# Autodesk Inventor assembly: Pod_pull
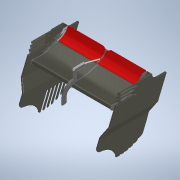
[picture p0: Inventor's stored thumbnail of the model, 180x180]
Saved by Autodesk Inventor 2022 (Build 260153000, 153)
## iProperties
Created: 2022-07-04
Part Number: Pod_pull
Document SubType Name: Assembly
Designer: corra
Author: corra
## Documents named in this file (7)
- C:\Users\corra\Desktop\Università Trento\Master degree\1st year\Mechatronic system simulation\Module 2\DRS_Project\File Cad 3D\final\assembly.iam
- C:\Users\corra\Desktop\Università Trento\Master degree\1st year\Mechatronic system simulation\Module 2\DRS_Project\File Cad 3D\final\flap.ipt
- C:\Users\corra\Desktop\Università Trento\Master degree\1st year\Mechatronic system simulation\Module 2\DRS_Project\File Cad 3D\final\main_plate.ipt
- C:\Users\corra\Desktop\Università Trento\Master degree\1st year\Mechatronic system simulation\Module 2\DRS_Project\File Cad 3D\final\pod.ipt
- C:\Users\corra\Desktop\Università Trento\Master degree\1st year\Mechatronic system simulation\Module 2\DRS_Project\File Cad 3D\final\actuator.ipt
- C:\Users\corra\Documents\Inventor\Content Center Files\R2022\it-IT\BS 1804\BS 1804-2 - 5 x 12.ipt
- C:\Users\corra\Documents\Inventor\Content Center Files\R2022\it-IT\BS 1804\BS 1804-2 - 3 x 10.ipt
## Components (6 placed, 6 different names)
1. flap:1 — Coincidente:1, Coincidente:2, Coincidente:4, Allineato:4, Coincidente:14, Coincidente:15, Allineato:5
2. main_plate:1 — Coincidente:1, Coincidente:2, Coincidente:5, Allineato:3, Coincidente:13
3. pod:1 — Coincidente:4, Coincidente:11, Coincidente:14
4. actuator:1 — Coincidente:5, Coincidente:10, Coincidente:12, Coincidente:13
5. BS 1804 : Parte 2 3 x 10:1 — Coincidente:10, Coincidente:11, Coincidente:12
6. BS 1804 : Parte 2 5 x 12:2 — Coincidente:15, Allineato:5
## Relationships (13: Mate 10, Flush 3)
- Coincidente:1 [Mate]: flap:1 ↔ main_plate:1
- Coincidente:2 [Mate]: flap:1 ↔ main_plate:1
- Coincidente:4 [Mate]: flap:1 ↔ pod:1
- Coincidente:5 [Mate]: main_plate:1 ↔ actuator:1
- Allineato:3 [Flush]: main_plate:1
- Allineato:4 [Flush]: flap:1
- Coincidente:10 [Mate]: actuator:1 ↔ BS 1804 : Parte 2 3 x 10:1
- Coincidente:11 [Mate]: pod:1 ↔ BS 1804 : Parte 2 3 x 10:1
- Coincidente:12 [Mate] (1.5 mm): actuator:1 ↔ BS 1804 : Parte 2 3 x 10:1
- Coincidente:13 [Mate]: main_plate:1 ↔ actuator:1
- Coincidente:14 [Mate]: flap:1 ↔ pod:1
- Coincidente:15 [Mate]: flap:1 ↔ BS 1804 : Parte 2 5 x 12:2
- Allineato:5 [Flush] (-1 mm): flap:1 ↔ BS 1804 : Parte 2 5 x 12:2
